# Autodesk Inventor assembly: Shifter Assembly
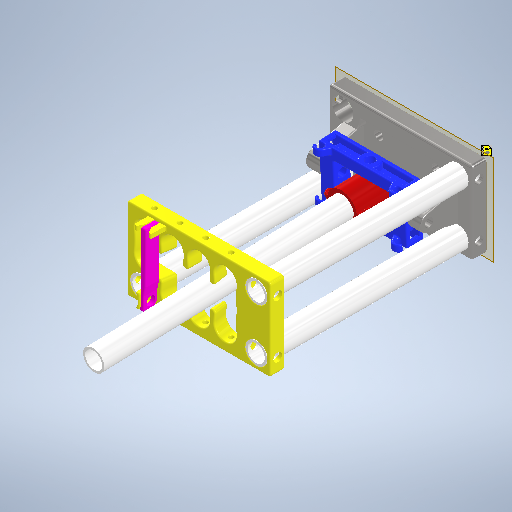
[picture p0: Inventor's stored thumbnail of the model, 512x512]
Saved by Autodesk Inventor 2025.2 (Build 292293000, 293)
## iProperties
Created: 2025-02-09
Part Number: Shifter Assembly
Document SubType Name: Assembly
Designer: eason
Author: eason
## Documents named in this file (8)
- C:\Users\eason\Desktop\Code\Unojoy-Simulator-Rig\CAD\Shifter\Shifter Assembly.iam
- C:\Users\eason\Desktop\Code\Unojoy-Simulator-Rig\CAD\Shifter\Shifter Joint 2.ipt
- C:\Users\eason\Desktop\Code\Unojoy-Simulator-Rig\CAD\Shifter\Shifter Joint.ipt
- C:\Users\eason\Desktop\Code\Unojoy-Simulator-Rig\CAD\Shifter\Shifter PVC.ipt
- C:\Users\eason\Desktop\Code\Unojoy-Simulator-Rig\CAD\Shifter\Shifter Support.ipt
- C:\Users\eason\Desktop\Code\Unojoy-Simulator-Rig\CAD\Shifter\Shifter Post.ipt
- C:\Users\eason\Desktop\Code\Unojoy-Simulator-Rig\CAD\Shifter\Shifter Gater.ipt
- C:\Users\eason\Desktop\Code\Unojoy-Simulator-Rig\CAD\Shifter\Reverse Lockout.ipt
## Components (9 placed, 7 different names)
1. Shifter Gater:1 — Cylindrical:8, Cylindrical:9, Mate:9, Cylindrical:14, Mate:18
2. Shifter Joint:1 — Cylindrical:3, Mate:15, Mate:16, Tangent:1
3. Shifter PVC:1 — Cylindrical:3, Mate:15
4. Shifter Post:1 — Cylindrical:13, Mate:17
5. Shifter Post:2 — Cylindrical:8, Mate:9, Cylindrical:11, Mate:13
6. Shifter Post:3 — Cylindrical:9, Cylindrical:10, Mate:12
7. Shifter Joint 2:1 — Cylindrical:12, Mate:14, Mate:16, Tangent:1
8. Shifter Support:1 — Mate:10, Mate:11, Cylindrical:10, Cylindrical:11, Mate:12, Mate:13, Cylindrical:12, Mate:14, Cylindrical:13, Mate:17
9. Reverse Lockout:1 — Cylindrical:14, Mate:18
## Relationships (19: Mate 10, CylindricalJoint 8, Tangent 1)
- Cylindrical:3: Shifter Joint:1 ↔ Shifter PVC:1
- Cylindrical:8: Shifter Gater:1 ↔ Shifter Post:2
- Cylindrical:9: Shifter Gater:1 ↔ Shifter Post:3
- Mate:9: Shifter Gater:1 ↔ Shifter Post:2
- Mate:10: Shifter Support:1
- Mate:11: Shifter Support:1
- Cylindrical:10: Shifter Post:3 ↔ Shifter Support:1
- Cylindrical:11: Shifter Post:2 ↔ Shifter Support:1
- Mate:12: Shifter Post:3 ↔ Shifter Support:1
- Mate:13: Shifter Post:2 ↔ Shifter Support:1
- Cylindrical:12: Shifter Joint 2:1 ↔ Shifter Support:1
- Mate:14: Shifter Joint 2:1 ↔ Shifter Support:1
- Mate:15: Shifter Joint:1 ↔ Shifter PVC:1
- Mate:16: Shifter Joint:1 ↔ Shifter Joint 2:1
- Tangent:1: Shifter Joint:1 ↔ Shifter Joint 2:1
- Cylindrical:13: Shifter Post:1 ↔ Shifter Support:1
- Mate:17: Shifter Post:1 ↔ Shifter Support:1
- Cylindrical:14: Shifter Gater:1 ↔ Reverse Lockout:1
- Mate:18: Shifter Gater:1 ↔ Reverse Lockout:1
